# Autodesk Inventor assembly: Motor_106
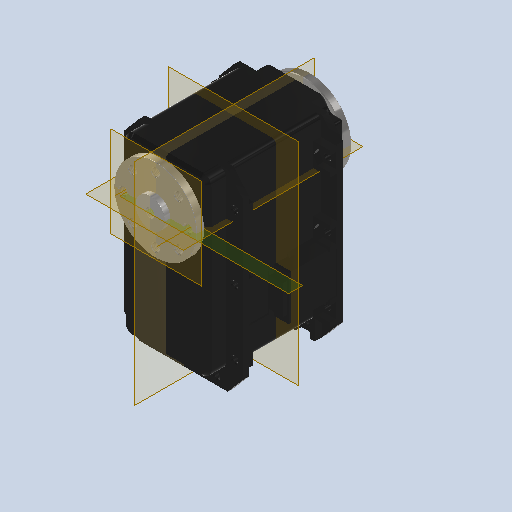
[picture p0: Inventor's stored thumbnail of the model, 512x512]
Saved by Autodesk Inventor 2024.3 (Build 283343000, 343)
## iProperties
Created: 2024-09-05
Part Number: Motor_106
Document SubType Name: Assembly
Designer: gretc
Author: gretc
## Documents named in this file (4)
- C:\Users\USER\Desktop\로빛 예비인턴\(git)19기 이원준 격투로봇 설계파일\motor\Motor_106.iam
- C:\Users\USER\Desktop\로빛 예비인턴\예비인턴 격투로봇 설계 프로젝트\격투로봇 백업 2\다이나믹셀\MX-106T+idle.ipt.iam
- C:\Users\USER\Desktop\로빛 예비인턴\예비인턴 격투로봇 설계 프로젝트\혼\64-106Horn.ipt
- MX-106T+idle.ipt
## Components (2 placed, 2 different names)
1. MX-106T+idle.ipt:1 [sub-assembly] — 삽입:1, 각도:1
2. 64-106Horn:1 — 삽입:1, 메이트:1, 메이트:2
## Relationships (4: Mate 2, Insert 1, Angle 1)
- 삽입:1 [Insert] (0.5 mm): MX-106T+idle.ipt:1 ↔ 64-106Horn:1
- 메이트:1 [Mate]: 64-106Horn:1
- 메이트:2 [Mate]: 64-106Horn:1
- 각도:1 [Angle] (90 deg): MX-106T+idle.ipt:1
